# Autodesk Inventor assembly: BBM Staging Plate Assembly
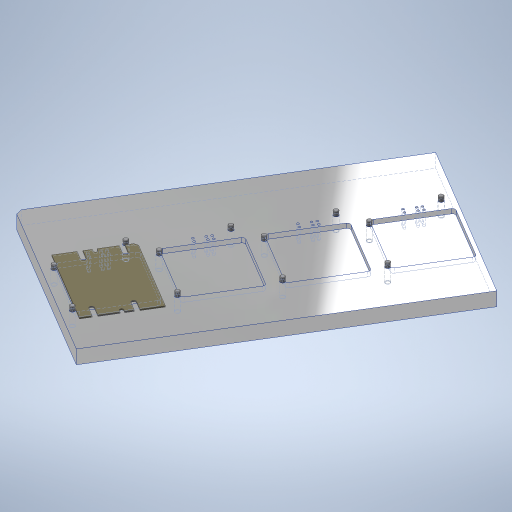
[picture p0: Inventor's stored thumbnail of the model, 512x512]
Saved by Autodesk Inventor 2023 (Build 270158000, 158)
## iProperties
Created: 2021-01-11
Part Number: BBM Staging Plate Assembly
Document SubType Name: Assembly
Designer: caleb
Author: caleb
## Documents named in this file (4)
- C:\Users\Caleb\Desktop\nebraska-silicon-lab\Hardware\ETL\Module Assembly\Baseplate Staging Plate - V3\Baseplate Staging Plate Assembly - V3.iam
- C:\Users\Caleb\Desktop\nebraska-silicon-lab\Hardware\ETL\Module Assembly\Baseplate Staging Plate - V3\Baseplate Staging Plate - V3.ipt
- C:\Users\Caleb\Desktop\nebraska-silicon-lab\Hardware\ETL\Module Assembly\Baseplate Staging Plate - V3\98381A304_Dowel Pin.ipt
- C:\Users\Caleb\Desktop\nebraska-silicon-lab\Hardware\ETL\modules\throughput mockups\Baseplate v1.5.ipt
## Components (14 placed, 3 different names)
1. Baseplate Staging Plate - V3:1 — Insert:1, Insert:2, Insert:3, Insert:4, Insert:5, Insert:6, Insert:7, Insert:8, Insert:9, Insert:10, Insert:11, Insert:12, Mate:1
2. 98381A304_Dowel Pin:1 — Insert:3, Tangent:1
3. 98381A304_Dowel Pin:2 — Insert:1, Tangent:3
4. 98381A304_Dowel Pin:3 — Insert:2, Tangent:2
5. 98381A304_Dowel Pin:4 — Insert:4
6. 98381A304_Dowel Pin:5 — Insert:5
7. 98381A304_Dowel Pin:6 — Insert:6
8. 98381A304_Dowel Pin:7 — Insert:7
9. 98381A304_Dowel Pin:8 — Insert:8
10. 98381A304_Dowel Pin:9 — Insert:9
11. 98381A304_Dowel Pin:10 — Insert:10
12. 98381A304_Dowel Pin:11 — Insert:11
13. 98381A304_Dowel Pin:12 — Insert:12
14. Baseplate v1.5:1 — Mate:1, Tangent:1, Tangent:2, Tangent:3
## Relationships (16: Insert 12, Tangent 3, Mate 1)
- Insert:1: Baseplate Staging Plate - V3:1 ↔ 98381A304_Dowel Pin:2
- Insert:2: Baseplate Staging Plate - V3:1 ↔ 98381A304_Dowel Pin:3
- Insert:3: Baseplate Staging Plate - V3:1 ↔ 98381A304_Dowel Pin:1
- Insert:4: Baseplate Staging Plate - V3:1 ↔ 98381A304_Dowel Pin:4
- Insert:5: Baseplate Staging Plate - V3:1 ↔ 98381A304_Dowel Pin:5
- Insert:6: Baseplate Staging Plate - V3:1 ↔ 98381A304_Dowel Pin:6
- Insert:7: Baseplate Staging Plate - V3:1 ↔ 98381A304_Dowel Pin:7
- Insert:8: Baseplate Staging Plate - V3:1 ↔ 98381A304_Dowel Pin:8
- Insert:9: Baseplate Staging Plate - V3:1 ↔ 98381A304_Dowel Pin:9
- Insert:10: Baseplate Staging Plate - V3:1 ↔ 98381A304_Dowel Pin:10
- Insert:11: Baseplate Staging Plate - V3:1 ↔ 98381A304_Dowel Pin:11
- Insert:12: Baseplate Staging Plate - V3:1 ↔ 98381A304_Dowel Pin:12
- Mate:1: Baseplate Staging Plate - V3:1 ↔ Baseplate v1.5:1
- Tangent:1: 98381A304_Dowel Pin:1 ↔ Baseplate v1.5:1
- Tangent:2: 98381A304_Dowel Pin:3 ↔ Baseplate v1.5:1
- Tangent:3: 98381A304_Dowel Pin:2 ↔ Baseplate v1.5:1
